# Autodesk Inventor assembly: XY Joint Left (Tulip)
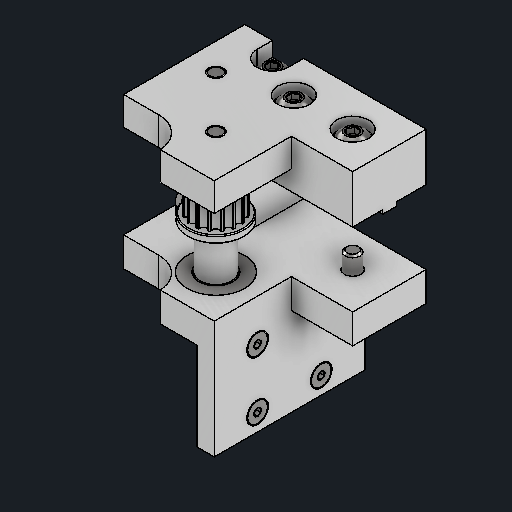
[picture p0: Inventor's stored thumbnail of the model, 512x512]
Saved by Autodesk Inventor 2026.1 (Build 301233020, 233B)
## iProperties
Created: 2025-05-24
Part Number: XY Joint Left (Tulip)
Document SubType Name: Assembly
Designer: Joshua Eah
Author: Joshua Eah
## Documents named in this file (10)
- C:\Users\JoshuaEah\Documents\GitHub\Voron-0\CAD\X Axis\XY Joints\XY Joint Left\XY Joint Left (Tulip).iam
- C:\Users\JoshuaEah\Documents\GitHub\Voron-0\CAD\X Axis\XY Joints\XY Joint Left\XY Joint Left Upper.ipt
- C:\Users\JoshuaEah\Documents\GitHub\Voron-0\CAD\X Axis\XY Joints\XY Joint Left\XY Joint Left Lower.ipt
- C:\Users\JoshuaEah\Documents\GitHub\Voron-0\CAD\Hardware\Fasteners\M3x6 BHCS.ipt
- C:\Users\JoshuaEah\Documents\GitHub\Voron-0\CAD\Hardware\Fasteners\M3x12 BHCS.ipt
- C:\Users\JoshuaEah\Documents\GitHub\Voron-0\CAD\Hardware\Fasteners\M2x6 FHCS.ipt
- C:\Users\JoshuaEah\Documents\GitHub\Voron-0\CAD\X Axis\XY Joints\Spacers\Joint Spacer.ipt
- C:\Users\JoshuaEah\Documents\GitHub\Voron-0\CAD\X Axis\XY Joints\XY Joint Left\Left Pulley Stack.iam
- C:\Users\JoshuaEah\Documents\GitHub\Voron-0\CAD\X Axis\XY Joints\XY Joint Left\Left Idler Stack.iam
- C:\Users\JoshuaEah\Documents\GitHub\Voron-0\CAD\Hardware\Fasteners\M3x25 BHCS.ipt
## Components (13 placed, 9 different names)
1. XY Joint Left Upper:1 — Insert:13, Insert:14, Insert:22, Mate:12, Insert:23
2. XY Joint Left Lower:1 — Insert:12, Insert:15, Insert:16, Insert:17, Insert:18, Insert:21
3. Left Pulley Stack:1 [sub-assembly]
4. Left Idler Stack:1 [sub-assembly]
5. M3x6 BHCS:1 — Insert:12
6. M3x12 BHCS:1 — Insert:13
7. M3x12 BHCS:2 — Insert:14
8. M2x6 FHCS:1 — Insert:15
9. M2x6 FHCS:2 — Insert:16
10. M2x6 FHCS:3 — Insert:17
11. M2x6 FHCS:4 — Insert:18
12. Joint Spacer:1 — Insert:21, Insert:22, Mate:12
13. M3x25 BHCS:1 — Insert:23
## Relationships (20: Insert 11, Mate 8, Flush 1)
- [Mate]: XY Joint Left Lower:1 ↔ Left Idler Stack:1
- [Mate]: XY Joint Left Lower:1 ↔ Left Idler Stack:1
- [Mate]: XY Joint Left Lower:1 ↔ Left Idler Stack:1
- Insert:12: XY Joint Left Lower:1 ↔ M3x6 BHCS:1
- Insert:13: XY Joint Left Upper:1 ↔ M3x12 BHCS:1
- Insert:14: XY Joint Left Upper:1 ↔ M3x12 BHCS:2
- Insert:15: XY Joint Left Lower:1 ↔ M2x6 FHCS:1
- Insert:16: XY Joint Left Lower:1 ↔ M2x6 FHCS:2
- Insert:17: XY Joint Left Lower:1 ↔ M2x6 FHCS:3
- Insert:18: XY Joint Left Lower:1 ↔ M2x6 FHCS:4
- [Insert]: XY Joint Left Upper:1 ↔ Left Idler Stack:1
- [Mate]: XY Joint Left Lower:1 ↔ Left Pulley Stack:1
- [Mate]: XY Joint Left Lower:1 ↔ Left Pulley Stack:1
- [Mate]: XY Joint Left Upper:1 ↔ Left Pulley Stack:1
- [Mate]: XY Joint Left Upper:1 ↔ Left Pulley Stack:1
- [Flush]: XY Joint Left Upper:1 ↔ Left Pulley Stack:1
- Insert:21: XY Joint Left Lower:1 ↔ Joint Spacer:1
- Insert:22: XY Joint Left Upper:1 ↔ Joint Spacer:1
- Mate:12: XY Joint Left Upper:1 ↔ Joint Spacer:1
- Insert:23: XY Joint Left Upper:1 ↔ M3x25 BHCS:1
